# Autodesk Inventor assembly: BaneBotWheel_MIR2
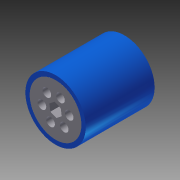
[picture p0: Inventor's stored thumbnail of the model, 180x180]
Saved by Autodesk Inventor 2012 (Build 160160000, 160)
## iProperties
Created: 2012-02-07
Part Number: BaneBotWheel_MIR2
Document SubType Name: Assembly
Designer: admin
Mass: 49.0421 g
Surface Area: 172.608 cm^2
Volume: 23.993 cm^3
Density: 2.04402 g/cm^3
Author: admin
## Documents named in this file (3)
- C:\Users\Admin\Documents\Inventor\SumoJaime2012\BaneBotWheel_MIR2.iam
- C:\Users\Admin\Documents\Inventor\SumoJaime2012\WheelTread_MIR1.ipt
- C:\Users\Admin\Documents\Inventor\SumoJaime2012\WheelHub_MIR1.ipt
## Components (2 placed, 2 different names)
1. WheelTread_MIR1:1 — Insert:1
2. WheelHub_MIR1:1 — Insert:1
## Relationships (1: Insert 1)
- Insert:1: WheelTread_MIR1:1 ↔ WheelHub_MIR1:1
